# Autodesk Inventor assembly: Manubrio_ruta
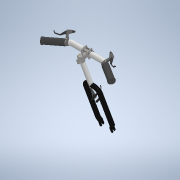
[picture p0: Inventor's stored thumbnail of the model, 180x180]
Saved by Autodesk Inventor 2021 (Build 250183000, 183)
## iProperties
Created: 2021-04-24
Part Number: Manubrio_ruta
Document SubType Name: Assembly
Designer: maaro
Author: maaro
## Documents named in this file (14)
- C:\Git\Proyecto_APM\02 Inventor\bicicleta_ruta\Manubrio\Manubrio_ruta.iam
- C:\Git\Proyecto_APM\02 Inventor\bicicleta_ruta\Manubrio\Mango Der.ipt
- C:\Git\Proyecto_APM\02 Inventor\bicicleta_ruta\Manubrio\Mango Izq.ipt
- C:\Git\Proyecto_APM\02 Inventor\bicicleta_ruta\Manubrio\Copa Tenedor.ipt
- C:\Git\Proyecto_APM\02 Inventor\bicicleta_ruta\Manubrio\Tubo Tenedor Izq.ipt
- C:\Git\Proyecto_APM\02 Inventor\bicicleta_ruta\Manubrio\Tubo Tenedor Der.ipt
- C:\Git\Proyecto_APM\02 Inventor\bicicleta_ruta\Manubrio\Tubo Tenedor Central.ipt
- C:\Git\Proyecto_APM\02 Inventor\bicicleta_ruta\Manubrio\Potencia Tras.ipt
- C:\Git\Proyecto_APM\02 Inventor\bicicleta_ruta\Manubrio\Potencia Del.ipt
- C:\Git\Proyecto_APM\02 Inventor\bicicleta_ruta\caña bici ruta.ipt
- C:\Git\Proyecto_APM\02 Inventor\bicicleta_ruta\Freno\FRENO\1 FRENO ENSAMBLADO.iam
- C:\Git\Proyecto_APM\02 Inventor\bicicleta_ruta\Freno\FRENO\1 FRENO ENSAMBLADO_MIR1.iam
- C:\Git\Proyecto_APM\02 Inventor\union_frenos.ipt
- C:\Git\Proyecto_APM\02 Inventor\bicicleta_ruta\Freno\BIKE V-BRAKE.iam
## Components (13 placed, 13 different names)
1. Mango Der:1 — Mate:2, Mate:4
2. Mango Izq:1 — Mate:3, Mate:5, Mate:7, Mate:10
3. Copa Tenedor:1
4. Tubo Tenedor Izq:1 — Mate:12
5. Tubo Tenedor Der:1 — Mate:11
6. Tubo Tenedor Central:1 — Mate:15
7. Potencia Tras:1 — Mate:1
8. Potencia Del:1 — Mate:6, Angle:1
9. caña bici ruta:1 — Mate:1, Mate:2, Mate:3, Mate:4, Mate:5, Mate:6, Angle:1
10. 1 FRENO ENSAMBLADO:1 [sub-assembly] — Mate:7, Mate:10
11. 1 FRENO ENSAMBLADO_MIR1:1 [sub-assembly]
12. union_frenos:1 — Flush:1, Flush:2, Rotational:1
13. BIKE V-BRAKE:1 [sub-assembly] — Rotational:1
## Relationships (17: Mate 13, Flush 2, Angle 1, RevoluteJoint 1)
- Mate:1: Potencia Tras:1 ↔ caña bici ruta:1
- Mate:2: Mango Der:1 ↔ caña bici ruta:1
- Mate:3: Mango Izq:1 ↔ caña bici ruta:1
- Mate:4: Mango Der:1 ↔ caña bici ruta:1
- Mate:5: Mango Izq:1 ↔ caña bici ruta:1
- Mate:6: Potencia Del:1 ↔ caña bici ruta:1
- Angle:1 (-10 deg): Potencia Del:1 ↔ caña bici ruta:1
- Mate:7: Mango Izq:1 ↔ 1 FRENO ENSAMBLADO:1
- Mate:10: Mango Izq:1 ↔ 1 FRENO ENSAMBLADO:1
- Mate:11: Tubo Tenedor Der:1
- Mate:12: Tubo Tenedor Izq:1
- Mate:13
- Mate:14
- Mate:15: Tubo Tenedor Central:1
- Flush:1: union_frenos:1
- Flush:2: union_frenos:1
- Rotational:1 [RevoluteJoint]: union_frenos:1 ↔ BIKE V-BRAKE:1
